# Autodesk Inventor assembly: SumoAssembly
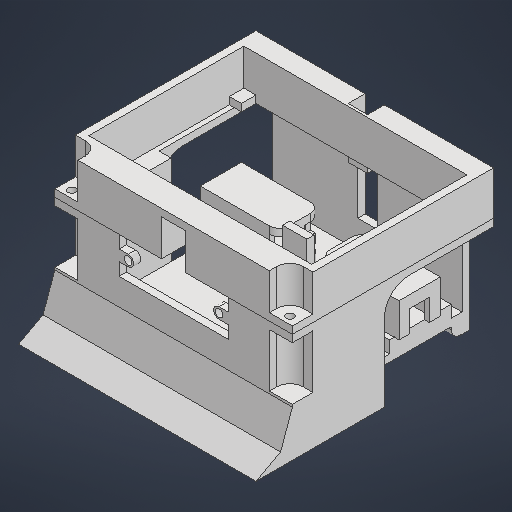
[picture p0: Inventor's stored thumbnail of the model, 512x512]
Saved by Autodesk Inventor 2026 (Build 300175000, 175)
## iProperties
Created: 2026-05-14
Part Number: SumoAssembly
Document SubType Name: Assembly
Designer: Patryk Lombardo
Author: Patryk Lombardo
## Documents named in this file (5)
- C:\Users\Patryk Lombardo\Desktop\programowanie\mikroprocesory\sumo\sumo_cad\SumoAssembly.iam
- C:\Users\Patryk Lombardo\Desktop\programowanie\mikroprocesory\sumo\sumo_cad\BodyBottom.ipt
- C:\Users\Patryk Lombardo\Desktop\programowanie\mikroprocesory\sumo\sumo_cad\BodyTop.ipt
- C:\Users\Patryk Lombardo\Desktop\programowanie\mikroprocesory\sumo\sumo_cad\EngineA.ipt
- C:\Users\Patryk Lombardo\Desktop\programowanie\mikroprocesory\sumo\sumo_cad\EngineB.ipt
## Components (4 placed, 4 different names)
1. BodyBottom:1 — Zestawiające:1, Zestawiające:2, Zestawiające:3, Zestawiające:4, Zestawiające:5, Zestawiające:6
2. BodyTop:1 — Zestawiające:1, Zestawiające:2
3. EngineA:1 — Zestawiające:3, Zestawiające:4
4. EngineB:1 — Zestawiające:5, Zestawiające:6
## Relationships (6: Mate 6)
- Zestawiające:1 [Mate]: BodyBottom:1 ↔ BodyTop:1
- Zestawiające:2 [Mate]: BodyBottom:1 ↔ BodyTop:1
- Zestawiające:3 [Mate]: BodyBottom:1 ↔ EngineA:1
- Zestawiające:4 [Mate]: BodyBottom:1 ↔ EngineA:1
- Zestawiające:5 [Mate]: BodyBottom:1 ↔ EngineB:1
- Zestawiające:6 [Mate]: BodyBottom:1 ↔ EngineB:1
